# Autodesk Inventor assembly: Lap-Corner-Brace
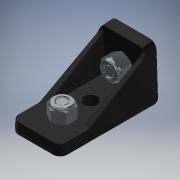
[picture p0: Inventor's stored thumbnail of the model, 180x180]
Saved by Autodesk Inventor 2017.3 (Build 213256000, 256)
## iProperties
Created: 2018-01-06
Part Number: Lap-Corner-Brace
Document SubType Name: Assembly
Designer: pranav
Author: pranav
## iProperties of the stored document REV-41-1359 Simple.ipt
Created: 2017-04-10
Part Number: REV-41-1359 Simple
Material: Generic
Document SubType Name: Modeling
Designer: pranav
Density: 1 g/cm^3
Appearance: Default
Sending System: Autodesk Translation Framework v5.2.0.2920
Preprocessor: ST-DEVELOPER v16.5
Title: E:/Dropbox/REV Robotics/STEP Files/REV-41-1359 Simple.step
## iProperties of the stored document REV-41-1321.ipt
Created: 2016-09-04
Part Number: REV-41-1321
Material: Generic
Description: STEP AP203
Document SubType Name: Modeling
Designer: pranav
Density: 1 g/cm^3
Appearance: Default
Sending System: SolidWorks 2015
Preprocessor: SwSTEP 2.0
Title: REV-41-1321_Default.step
Revision Number: ANY
## iProperties of the stored document REV-41-1361 Simple.ipt
Created: 2017-04-10
Part Number: REV-41-1361 Simple
Material: Generic
Document SubType Name: Modeling
Designer: pranav
Density: 1 g/cm^3
Appearance: Default
Sending System: Autodesk Translation Framework v5.2.0.2920
Preprocessor: ST-DEVELOPER v16.5
Title: E:/Dropbox/REV Robotics/STEP Files/REV-41-1361 Simple.step
## Documents named in this file (7)
- **C:\Users\pranav\Documents\Inventor\REV-Robot-CAD\Lap-Corner-Brace.iam*LocalDocs*xIq20mfpjXxsgews0Ysoywho13g*REV-41-1359 Simple.ipt
- **C:\Users\pranav\Documents\Inventor\REV-Robot-CAD\Lap-Corner-Brace.iam*LocalDocs*x5cc0c4chXm0cexkpAidds3vwHf*REV-41-1321.ipt
- **C:\Users\pranav\Documents\Inventor\REV-Robot-CAD\Lap-Corner-Brace.iam*LocalDocs*xKark4dgf5cu3upoeKvpt0vvzEh*REV-41-1361 Simple.ipt
- C:\Users\pranav\Documents\Inventor\REV-Robot-CAD\Lap-Corner-Brace.iam
- C:\Users\pranav\Documents\Inventor\REV-Robot-CAD\REV Robotics\REV Robotics CAD\REV-41-1321.step
- C:\Users\pranav\Documents\Inventor\REV-Robot-CAD\REV Robotics\REV Robotics CAD\REV-41-1359 Simple.step
- C:\Users\pranav\Documents\Inventor\REV-Robot-CAD\REV Robotics\REV Robotics CAD\REV-41-1361 Simple.step
## Components (5 placed, 3 different names)
1. REV-41-1321:1 — Mate:5, Mate:7, Mate:8, Mate:9
2. REV-41-1359 Simple:1 — Mate:7, Mate:10
3. REV-41-1359 Simple:2 — Mate:5, Mate:11
4. REV-41-1361 Simple:1 — Mate:8, Mate:10
5. REV-41-1361 Simple:2 — Mate:9, Mate:11
## Relationships (6: Mate 6)
- Mate:5: REV-41-1321:1 ↔ REV-41-1359 Simple:2
- Mate:7: REV-41-1321:1 ↔ REV-41-1359 Simple:1
- Mate:8: REV-41-1321:1 ↔ REV-41-1361 Simple:1
- Mate:9: REV-41-1321:1 ↔ REV-41-1361 Simple:2
- Mate:10: REV-41-1359 Simple:1 ↔ REV-41-1361 Simple:1
- Mate:11: REV-41-1359 Simple:2 ↔ REV-41-1361 Simple:2
